# Autodesk Inventor assembly: ElectronGun
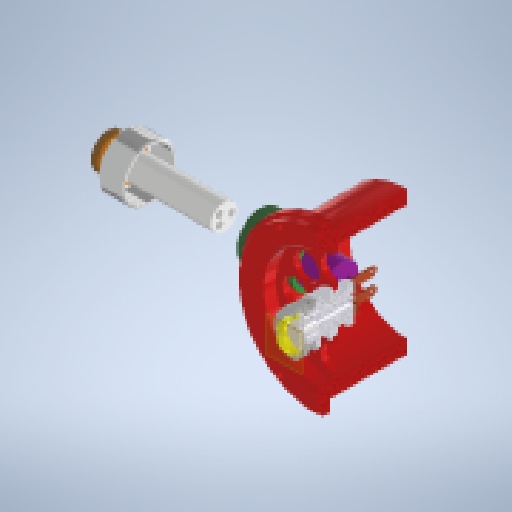
[picture p0: Inventor's stored thumbnail of the model, 512x512]
Saved by Autodesk Inventor 2023 (Build 270158000, 158)
## iProperties
Created: 2022-03-31
Part Number: ElectronGun
Document SubType Name: Assembly
Designer: Vinicius Miguel
Mass: 2242.74 g
Surface Area: 1358.94 cm^2
Volume: 426.533 cm^3
Density: 5.25806 g/cm^3
Author: Vinicius Miguel
## Documents named in this file (13)
- P:\SEM-Mechanical\ElectronGun.iam
- P:\SEM-Mechanical\016.ipt
- P:\SEM-Mechanical\017.ipt
- P:\SEM-Mechanical\018.ipt
- P:\SEM-Mechanical\021.ipt
- P:\SEM-Mechanical\027.ipt
- P:\SEM-Mechanical\028.ipt
- P:\SEM-Mechanical\029.ipt
- P:\SEM-Mechanical\030.ipt
- P:\SEM-Mechanical\031.ipt
- P:\SEM-Mechanical\Filament.ipt
- P:\SEM-Mechanical\032.ipt
- P:\SEM-Mechanical\033.ipt
## Components (13 placed, 12 different names)
1. 016:1 — Mate:1, Mate:2, Mate:3, Rotational:3, Mate:10
2. 017:1 — Rotational:3
3. 018:1 — Mate:4, Mate:9, Rotational:12
4. 021:1 — Mate:6, Mate:8, Rotational:6, Angle:3, Rotational:11
5. 027:1 — Rotational:5, Rotational:6
6. 028:1 — Rotational:5, Angle:1, Angle:2, Angle:3
7. 029:1 — Rotational:8
8. 030:1 — Rotational:8, Rotational:10
9. 031:1 — Rotational:10
10. Filament:1 — Mate:9, Mate:10
11. 032:1 — Angle:1, Flush:1
12. 032:2 — Angle:2, Flush:1
13. 033:1 — Rotational:11, Rotational:12
## Relationships (19: Mate 8, RevoluteJoint 7, Angle 3, Flush 1)
- Mate:1: 016:1
- Mate:2: 016:1
- Mate:3: 016:1
- Mate:4: 018:1
- Mate:6: 021:1
- Rotational:3 [RevoluteJoint]: 016:1 ↔ 017:1
- Rotational:5 [RevoluteJoint]: 027:1 ↔ 028:1
- Mate:8: 021:1
- Rotational:6 [RevoluteJoint]: 021:1 ↔ 027:1
- Rotational:8 [RevoluteJoint]: 029:1 ↔ 030:1
- Rotational:10 [RevoluteJoint]: 030:1 ↔ 031:1
- Mate:9: 018:1 ↔ Filament:1
- Mate:10: 016:1 ↔ Filament:1
- Angle:1 (180 deg): 028:1 ↔ 032:1
- Angle:2 (180 deg): 028:1 ↔ 032:2
- Flush:1: 032:1 ↔ 032:2
- Angle:3 (0 deg): 021:1 ↔ 028:1
- Rotational:11 [RevoluteJoint]: 021:1 ↔ 033:1
- Rotational:12 [RevoluteJoint]: 018:1 ↔ 033:1
